# Autodesk Inventor assembly: Frame
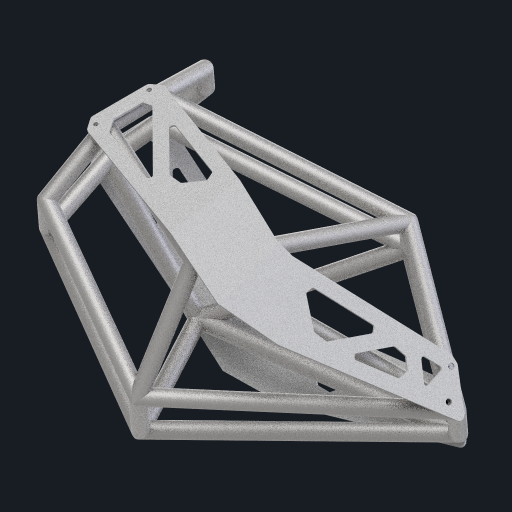
[picture p0: Inventor's stored thumbnail of the model, 512x512]
Saved by Autodesk Inventor 2023 (Build 270158000, 158)
## iProperties
Created: 2023-12-08
Part Number: Frame
Document SubType Name: Assembly
Designer: valer
_FrameDoc: Frame Assembly
_Version: 15.0.0
Author: valer
## Documents named in this file (31)
- C:\Users\valer\Desktop\str1ker\cad\chest\Chest.iam
- C:\Users\valer\Desktop\str1ker\cad\chest\Skeleton.ipt
- C:\Users\valer\Desktop\str1ker\cad\chest\ANSI 1_2 x 0.147 1702054336438.ipt
- C:\Users\valer\Desktop\str1ker\cad\chest\ANSI 1_2 x 0.147 1702054336462.ipt
- C:\Users\valer\Desktop\str1ker\cad\chest\ANSI 1_2 x 0.147 1702054336487.ipt
- C:\Users\valer\Desktop\str1ker\cad\chest\ANSI 1_2 x 0.147 1702054336518.ipt
- C:\Users\valer\Desktop\str1ker\cad\chest\ANSI 1_2 x 0.147 1702054336542.ipt
- C:\Users\valer\Desktop\str1ker\cad\chest\ANSI 1_2 x 0.147 1702054336566.ipt
- C:\Users\valer\Desktop\str1ker\cad\chest\ANSI 1_2 x 0.147 1702054336590.ipt
- C:\Users\valer\Desktop\str1ker\cad\chest\ANSI 1_2 x 0.147 1702054336614.ipt
- C:\Users\valer\Desktop\str1ker\cad\chest\ANSI 1_2 x 0.147 1702054336638.ipt
- C:\Users\valer\Desktop\str1ker\cad\chest\ANSI 1_2 x 0.147 1702054336662.ipt
- C:\Users\valer\Desktop\str1ker\cad\chest\ANSI 1_2 x 0.147 1702054336691.ipt
- C:\Users\valer\Desktop\str1ker\cad\chest\ANSI 1_2 x 0.147 1702054336715.ipt
- C:\Users\valer\Desktop\str1ker\cad\chest\ANSI 1_2 x 0.147 1702054336739.ipt
- C:\Users\valer\Desktop\str1ker\cad\chest\ANSI 1_2 x 0.147 1702054336764.ipt
- C:\Users\valer\Desktop\str1ker\cad\chest\ANSI 1_2 x 0.147 1702054336787.ipt
- C:\Users\valer\Desktop\str1ker\cad\chest\ANSI 1_2 x 0.147 1702054336811.ipt
- C:\Users\valer\Desktop\str1ker\cad\chest\ANSI 1_2 x 0.147 1702054336842.ipt
- C:\Users\valer\Desktop\str1ker\cad\chest\ANSI 1_2 x 0.147 1702054336866.ipt
- C:\Users\valer\Desktop\str1ker\cad\chest\ANSI 1_2 x 0.147 1702054336890.ipt
- C:\Users\valer\Desktop\str1ker\cad\chest\ANSI 1_2 x 0.147 1702054336914.ipt
- C:\Users\valer\Desktop\str1ker\cad\chest\ANSI 1_2 x 0.147 1702054336937.ipt
- C:\Users\valer\Desktop\str1ker\cad\chest\ANSI 1_2 x 0.147 1702054336961.ipt
- C:\Users\valer\Desktop\str1ker\cad\chest\ANSI 1_2 x 0.147 1702054336987.ipt
- C:\Users\valer\Desktop\str1ker\cad\chest\ANSI 1_2 x 0.147 1702054337011.ipt
- C:\Users\valer\Desktop\str1ker\cad\chest\ANSI 1_2 x 0.147 1702054337036.ipt
- C:\Users\valer\Desktop\str1ker\cad\chest\ANSI 1_2 x 0.147 1702054337060.ipt
- C:\Users\valer\Desktop\str1ker\cad\chest\ANSI 1_2 x 0.147 1702054337084.ipt
- C:\Users\valer\Desktop\str1ker\cad\chest\ChestSide.ipt
- C:\Users\valer\Desktop\str1ker\cad\chest\ChestSideMirror1.ipt
## Components (30 placed, 19 different names)
1. Reference Skeleton
2. ANSI 1/2 x 0.147 - 12.219:1 — Mate:4
3. ANSI 1/2 x 0.147 - 10.633:1
4. ANSI 1/2 x 0.147 - 8.798:1 — Mate:5, Flush:3
5. ANSI 1/2 x 0.147 - 6.95:1
6. ANSI 1/2 x 0.147 - 12.219:2 — Mate:2
7. ANSI 1/2 x 0.147 - 8.798:2 — Mate:1
8. ANSI 1/2 x 0.147 - 6.428:1
9. ANSI 1/2 x 0.147 - 14.125:1
10. ANSI 1/2 x 0.147 - 14.125:2
11. ANSI 1/2 x 0.147 - 4.331:1
12. ANSI 1/2 x 0.147 - 2.824:1
13. ANSI 1/2 x 0.147 - 4.331:2 — Flush:2
14. ANSI 1/2 x 0.147 - 2.824:2 — Flush:1
15. ANSI 1/2 x 0.147 - 3.03:1
16. ANSI 1/2 x 0.147 - 4.876:1
17. ANSI 1/2 x 0.147 - 3.03:2
18. ANSI 1/2 x 0.147 - 7.403:1
19. ANSI 1/2 x 0.147 - 7.133:1
20. ANSI 1/2 x 0.147 - 9.922:1
21. ANSI 1/2 x 0.147 - 7.133:2
22. ANSI 1/2 x 0.147 - 13.839:1 — Mate:6, Flush:4
23. ANSI 1/2 x 0.147 - 8.474:1
24. ANSI 1/2 x 0.147 - 9.199:1
25. ANSI 1/2 x 0.147 - 10.633:2
26. ANSI 1/2 x 0.147 - 8.474:2
27. ANSI 1/2 x 0.147 - 9.922:2
28. ANSI 1/2 x 0.147 - 13.839:2 — Mate:3
29. ChestSide:1 — Flush:1, Flush:2, Flush:3, Flush:4
30. ChestSideMirror1:1
## Relationships (11: Mate 6, Flush 4, Symmetry 1)
- Mate:1: ANSI 1/2 x 0.147 - 8.798:2
- Mate:2: ANSI 1/2 x 0.147 - 12.219:2
- Mate:3: ANSI 1/2 x 0.147 - 13.839:2
- Mate:4: ANSI 1/2 x 0.147 - 12.219:1
- Mate:5: ANSI 1/2 x 0.147 - 8.798:1
- Mate:6: ANSI 1/2 x 0.147 - 13.839:1
- Symmetry:1
- Flush:1: ANSI 1/2 x 0.147 - 2.824:2 ↔ ChestSide:1
- Flush:2: ANSI 1/2 x 0.147 - 4.331:2 ↔ ChestSide:1
- Flush:3: ANSI 1/2 x 0.147 - 8.798:1 ↔ ChestSide:1
- Flush:4: ANSI 1/2 x 0.147 - 13.839:1 ↔ ChestSide:1
